# Autodesk Inventor assembly: Gyro Assembly
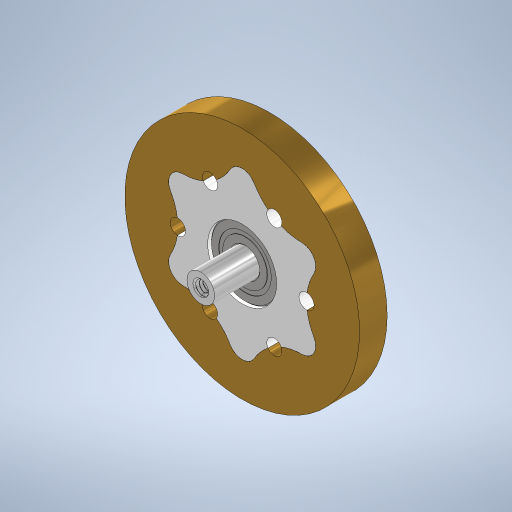
[picture p0: Inventor's stored thumbnail of the model, 512x512]
Saved by Autodesk Inventor 2023.2 (Build 272271000, 271)
## iProperties
Created: 2023-06-11
Part Number: Gyro Assembly
Document SubType Name: Assembly
Designer: Nathan Cai
Mass: 86.1562 g
Surface Area: 95.2051 cm^2
Volume: 14.2393 cm^3
Density: 6.05059 g/cm^3
Author: Nathan Cai
## Documents named in this file (5)
- E:\Documents\Inventor\Law - V1.0\Gyro Assembly.iam
- E:\Documents\Inventor\Law - V1.0\Brass Gryo.ipt
- E:\Documents\Inventor\Law - V1.0\5-8in OD Ball Bearing.ipt
- E:\Documents\Inventor\Law - V1.0\Gyro Core.ipt
- E:\Documents\Inventor\Law - V1.0\Standoff 1in.ipt
## Components (4 placed, 4 different names)
1. Brass Gryo:1 — Mate:1, Flush:1, Mate:3, Flush:2
2. 5-8in OD Ball Bearing:1 — Mate:1, Flush:1, Mate:2, Mate:4
3. Gyro Core:1 — Mate:2, Mate:3, Flush:2, Flush:3
4. Standoff 1in:1 — Mate:4, Flush:3
## Relationships (7: Mate 4, Flush 3)
- Mate:1: Brass Gryo:1 ↔ 5-8in OD Ball Bearing:1
- Flush:1 (0.635 mm): Brass Gryo:1 ↔ 5-8in OD Ball Bearing:1
- Mate:2: 5-8in OD Ball Bearing:1 ↔ Gyro Core:1
- Mate:3: Brass Gryo:1 ↔ Gyro Core:1
- Flush:2: Brass Gryo:1 ↔ Gyro Core:1
- Mate:4: 5-8in OD Ball Bearing:1 ↔ Standoff 1in:1
- Flush:3 (-9.525 mm): Gyro Core:1 ↔ Standoff 1in:1
